# Autodesk Inventor assembly: Top layer
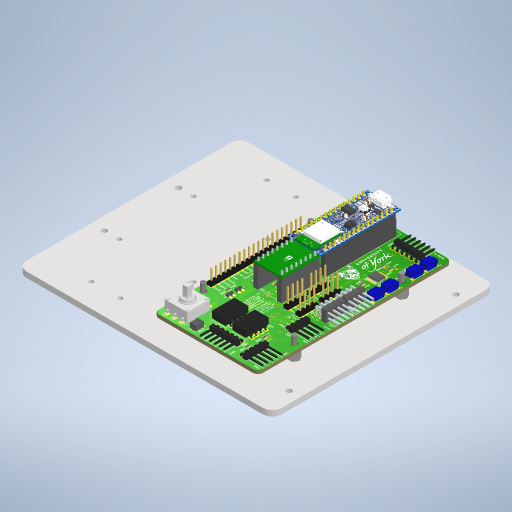
[picture p0: Inventor's stored thumbnail of the model, 512x512]
Saved by Autodesk Inventor 2023 (Build 270158000, 158)
## iProperties
Created: 2024-10-04
Part Number: Top layer
Document SubType Name: Assembly
Designer: bw1293
Author: bw1293
## Documents named in this file (5)
- \\userfs\bw1293\w2k\Inventor\Bw RDAC 1\Top layer.iam
- \\userfs\bw1293\w2k\Inventor\Bw RDAC 1\Top Layer.ipt
- \\userfs\bw1293\w2k\Inventor\Bw RDAC 1\ARB Board CAD model.ipt
- \\userfs\bw1293\w2k\Inventor\Bw RDAC 1\M2.5 Hex Spacer 5mm.ipt
- \\userfs\bw1293\w2k\Inventor\Bw RDAC 1\Top base 2.ipt
## Components (7 placed, 4 different names)
1. Top Layer:1
2. ARB Board CAD model:1 — Insert:1, Insert:2, Insert:4
3. M2.5 Hex Spacer 5mm:1 — Insert:4, Insert:5
4. M2.5 Hex Spacer 5mm:2 — Insert:7
5. M2.5 Hex Spacer 5mm:3 — Insert:2, Insert:8
6. M2.5 Hex Spacer 5mm:4 — Insert:1, Insert:6
7. Top base 2:1 — Insert:5, Insert:6, Insert:7, Insert:8
## Relationships (7: Insert 7)
- Insert:1: ARB Board CAD model:1 ↔ M2.5 Hex Spacer 5mm:4
- Insert:2: ARB Board CAD model:1 ↔ M2.5 Hex Spacer 5mm:3
- Insert:4: ARB Board CAD model:1 ↔ M2.5 Hex Spacer 5mm:1
- Insert:5: M2.5 Hex Spacer 5mm:1 ↔ Top base 2:1
- Insert:6: M2.5 Hex Spacer 5mm:4 ↔ Top base 2:1
- Insert:7: M2.5 Hex Spacer 5mm:2 ↔ Top base 2:1
- Insert:8: M2.5 Hex Spacer 5mm:3 ↔ Top base 2:1
